# Autodesk Inventor assembly: Bed Assembly
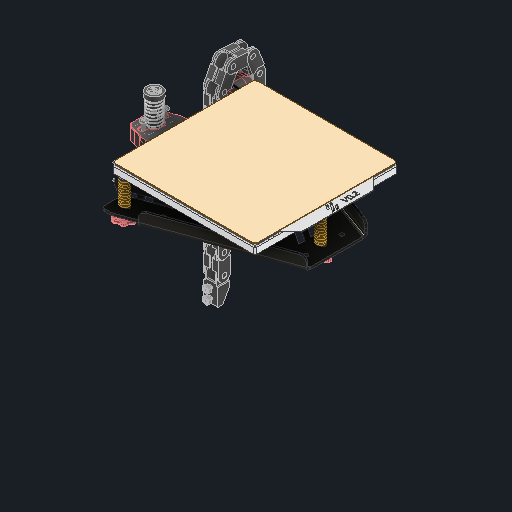
[picture p0: Inventor's stored thumbnail of the model, 512x512]
Saved by Autodesk Inventor 2025.1 (Build 291241020, 241B)
## iProperties
Created: 2025-05-09
Part Number: Bed Assembly
Document SubType Name: Assembly
Designer: AdminForWorker
Title: Bed Assembly
Author: AdminForWorker
## Documents named in this file (13)
- C:\Users\Joshua Eah\Documents\Voron 0.2\CAD\Master Assembly\Bed Assembly.iam
- C:\Users\Joshua Eah\Documents\Voron 0.2\CAD\Master Assembly\Build Plate.iam
- C:\Users\Joshua Eah\Documents\Voron 0.2\CAD\Master Assembly\Thumb Nuts.iam
- C:\Users\Joshua Eah\Documents\Voron 0.2\CAD\Master Assembly\IGUS Drag Chain.iam
- C:\Users\Joshua Eah\Documents\Voron 0.2\CAD\Master Assembly\Z Axis\Bed Assembly\Kirigami Bed.iam
- C:\Users\Joshua Eah\Documents\Voron 0.2\CAD\Master Assembly\Hardware\M3x16 BHCS.ipt
- C:\Users\Joshua Eah\Documents\Voron 0.2\CAD\Master Assembly\Hardware\M3x6 BHCS.ipt
- C:\Users\Joshua Eah\Documents\Voron 0.2\CAD\Master Assembly\Hardware\M3 Hexnut.ipt
- C:\Users\Joshua Eah\Documents\Voron 0.2\CAD\Master Assembly\Washers (4).iam
- C:\Users\Joshua Eah\Documents\Voron 0.2\CAD\Master Assembly\Springs.iam
- C:\Users\Joshua Eah\Documents\Voron 0.2\CAD\Master Assembly\Hardware\M3x40 BHCS.ipt
- C:\Users\Joshua Eah\Documents\Voron 0.2\CAD\Master Assembly\Hardware\M3x12 BHCS.ipt
- C:\Users\Joshua Eah\Documents\Voron 0.2\CAD\Master Assembly\TR8x8 Antibacklash Nut.ipt
## Components (21 placed, 12 different names)
1. Build Plate:1 [sub-assembly]
2. Thumb Nuts:1 [sub-assembly]
3. IGUS Drag Chain:1 [sub-assembly] — Insert:1, Insert:2, Insert:3, Insert:4, Insert:5, Insert:6
4. Kirigami Bed:1 [sub-assembly] — Insert:1, Insert:2
5. M3x16 BHCS:1 — Insert:3
6. M3x16 BHCS:2 — Insert:4
7. M3x6 BHCS:1 — Mate:3, Insert:5
8. M3x6 BHCS:2 — Mate:4, Insert:6
9. M3 Hexnut:1 — Mate:3
10. M3 Hexnut:2 — Mate:4
11. Washers (4):1 [sub-assembly]
12. Springs:1 [sub-assembly]
13. M3x40 BHCS:1
14. M3x40 BHCS:2
15. M3x40 BHCS:3
16. M3x12 BHCS:1
17. M3x12 BHCS:2
18. TR8x8 Antibacklash Nut:1
19. M3 Hexnut:3
20. M3 Hexnut:4
21. M3 Hexnut:5
## Relationships (10: Insert 6, Mate 4)
- [Mate]: Kirigami Bed:1 ↔ M3x40 BHCS:3
- [Mate]: Kirigami Bed:1 ↔ Springs:1
- Insert:1: IGUS Drag Chain:1 ↔ Kirigami Bed:1
- Insert:2: IGUS Drag Chain:1 ↔ Kirigami Bed:1
- Insert:3: IGUS Drag Chain:1 ↔ M3x16 BHCS:1
- Insert:4: IGUS Drag Chain:1 ↔ M3x16 BHCS:2
- Mate:3: M3x6 BHCS:1 ↔ M3 Hexnut:1
- Mate:4: M3x6 BHCS:2 ↔ M3 Hexnut:2
- Insert:5: IGUS Drag Chain:1 ↔ M3x6 BHCS:1
- Insert:6: IGUS Drag Chain:1 ↔ M3x6 BHCS:2
